# Autodesk Inventor assembly: main_rename
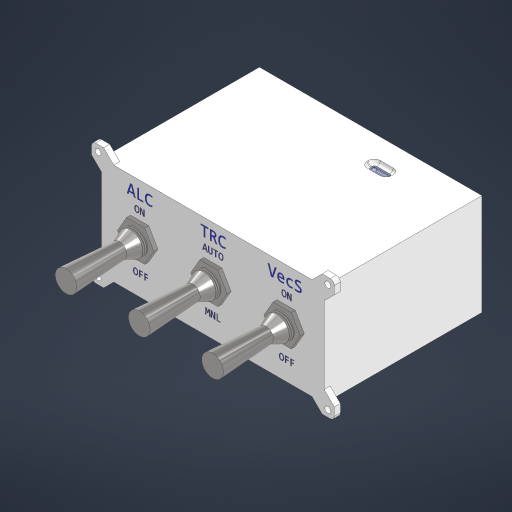
[picture p0: Inventor's stored thumbnail of the model, 512x512]
Saved by Autodesk Inventor 2024 (Build 280153000, 153)
## iProperties
Created: 2026-04-07
Part Number: main_rename
Document SubType Name: Assembly
Designer: schar
Author: schar
## Documents named in this file (7)
- C:\Users\schar\Desktop\MHIPS\models\tiles\2x1\lvl202x01_t\lvl202x01.iam
- C:\Users\schar\Desktop\MHIPS\models\tiles\2x1\lvl202x01_t\lvl202x01_toggle_body.ipt
- C:\Users\schar\Desktop\MHIPS\models\switches\NKK_S1AL.ipt
- C:\Users\schar\Desktop\MHIPS\models\switches\lvl2_2x2_guard.ipt
- C:\Users\schar\Desktop\MHIPS\models\BusPlate\BusPlate.iam
- C:\Users\schar\Desktop\MHIPS\models\tiles\2x1\lvl202x01_t\backplate_lvl202x01.ipt
- C:\Users\schar\Desktop\MHIPS\models\switches\NKK_S1AL_mother.ipt
## Components (10 placed, 6 different names)
1. lvl202x01_toggle_body:1 — Mate:1, Mate:2, Angle:1, Mate:3, Mate:4, Mate:5, Mate:6, Angle:2, Angle:3, Flush:2, Mate:7, Mate:8, Flush:3, Flush:6, Flush:7, Angle:4, Angle:5, Angle:6, Mate:11, Mate:12
2. NKK_S1AL:1 — Mate:1, Mate:2, Angle:1
3. NKK_S1AL:2 — Mate:4, Mate:6, Angle:3, Mate:10
4. NKK_S1AL:3 — Mate:3, Mate:5, Angle:2, Mate:9
5. lvl2_2x2_guard:1 — Flush:2
6. BusPlate:1 [sub-assembly] — Mate:7, Mate:8, Flush:4
7. backplate_lvl202x01:1 — Flush:3, Flush:4, Flush:5
8. NKK_S1AL_mother:1 — Flush:7, Angle:6
9. NKK_S1AL_mother:2 — Mate:10, Angle:5, Mate:11
10. NKK_S1AL_mother:3 — Mate:9, Angle:4, Mate:12
## Relationships (24: Mate 12, Angle 6, Flush 6)
- Mate:1: lvl202x01_toggle_body:1 ↔ NKK_S1AL:1
- Mate:2: lvl202x01_toggle_body:1 ↔ NKK_S1AL:1
- Angle:1 (0 deg): lvl202x01_toggle_body:1 ↔ NKK_S1AL:1
- Mate:3: lvl202x01_toggle_body:1 ↔ NKK_S1AL:3
- Mate:4: lvl202x01_toggle_body:1 ↔ NKK_S1AL:2
- Mate:5: lvl202x01_toggle_body:1 ↔ NKK_S1AL:3
- Mate:6: lvl202x01_toggle_body:1 ↔ NKK_S1AL:2
- Angle:2 (0 deg): lvl202x01_toggle_body:1 ↔ NKK_S1AL:3
- Angle:3 (0 deg): lvl202x01_toggle_body:1 ↔ NKK_S1AL:2
- Flush:2: lvl202x01_toggle_body:1 ↔ lvl2_2x2_guard:1
- Mate:7 (0.2 mm): lvl202x01_toggle_body:1 ↔ BusPlate:1
- Mate:8 (0.2 mm): lvl202x01_toggle_body:1 ↔ BusPlate:1
- Flush:3: lvl202x01_toggle_body:1 ↔ backplate_lvl202x01:1
- Flush:4: BusPlate:1 ↔ backplate_lvl202x01:1
- Flush:5: backplate_lvl202x01:1
- Flush:6: lvl202x01_toggle_body:1
- Flush:7: lvl202x01_toggle_body:1 ↔ NKK_S1AL_mother:1
- Mate:9: NKK_S1AL:3 ↔ NKK_S1AL_mother:3
- Mate:10: NKK_S1AL:2 ↔ NKK_S1AL_mother:2
- Angle:4 (0 deg): lvl202x01_toggle_body:1 ↔ NKK_S1AL_mother:3
- Angle:5 (0 deg): lvl202x01_toggle_body:1 ↔ NKK_S1AL_mother:2
- Angle:6 (0 deg): lvl202x01_toggle_body:1 ↔ NKK_S1AL_mother:1
- Mate:11: lvl202x01_toggle_body:1 ↔ NKK_S1AL_mother:2
- Mate:12: lvl202x01_toggle_body:1 ↔ NKK_S1AL_mother:3
